# Autodesk Inventor assembly: Ensamblaje Bomba
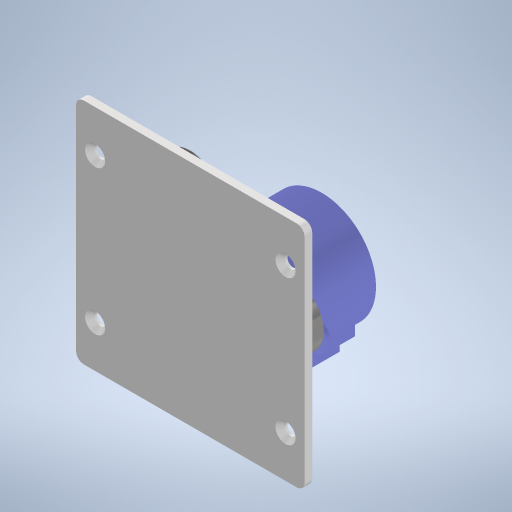
[picture p0: Inventor's stored thumbnail of the model, 512x512]
Saved by Autodesk Inventor 2023 (Build 270158000, 158)
## iProperties
Created: 2023-04-01
Part Number: Ensamblaje Bomba
Document SubType Name: Assembly
Designer: sergi
Author: sergi
## Documents named in this file (7)
- C:\Users\sergi\OneDrive\Escritorio\Objetos 3d\Bomba Persitaltica\Ensamblaje Bomba.iam
- C:\Users\sergi\OneDrive\Escritorio\Objetos 3d\Bomba Persitaltica\Imported Components\stepper_28byj-48\stepper_28byj-48.ipt
- C:\Users\sergi\OneDrive\Escritorio\Objetos 3d\Bomba Persitaltica\Soporte rodamientos.ipt
- C:\Users\sergi\OneDrive\Escritorio\Objetos 3d\Bomba Persitaltica\Rodamiento.ipt
- C:\Users\sergi\OneDrive\Escritorio\Objetos 3d\Bomba Persitaltica\Tapa Soporte rodamientos.ipt
- C:\Users\sergi\OneDrive\Escritorio\Objetos 3d\Bomba Persitaltica\Base.ipt
- C:\Users\sergi\OneDrive\Escritorio\Objetos 3d\Bomba Persitaltica\Tapa.ipt
## Components (8 placed, 6 different names)
1. stepper_28byj-48:1 — Coincidencia:9
2. Soporte rodamientos:1 — Coincidencia:5, Coincidencia:6, Coincidencia:7, Nivelación:1, Nivelación:2, Nivelación:3, Coincidencia:8, Coincidencia:10
3. Rodamiento:1 — Coincidencia:7, Nivelación:1
4. Rodamiento:2 — Coincidencia:5, Nivelación:2
5. Rodamiento:3 — Coincidencia:6, Nivelación:3
6. Tapa Soporte rodamientos:1 — Coincidencia:8
7. Base:1 — Coincidencia:9, Coincidencia:10, Nivelación:4
8. Tapa:1 — Nivelación:4
## Relationships (10: Mate 6, Flush 4)
- Coincidencia:5 [Mate]: Soporte rodamientos:1 ↔ Rodamiento:2
- Coincidencia:6 [Mate]: Soporte rodamientos:1 ↔ Rodamiento:3
- Coincidencia:7 [Mate]: Soporte rodamientos:1 ↔ Rodamiento:1
- Nivelación:1 [Flush]: Soporte rodamientos:1 ↔ Rodamiento:1
- Nivelación:2 [Flush]: Soporte rodamientos:1 ↔ Rodamiento:2
- Nivelación:3 [Flush]: Soporte rodamientos:1 ↔ Rodamiento:3
- Coincidencia:8 [Mate]: Soporte rodamientos:1 ↔ Tapa Soporte rodamientos:1
- Coincidencia:9 [Mate]: stepper_28byj-48:1 ↔ Base:1
- Coincidencia:10 [Mate]: Soporte rodamientos:1 ↔ Base:1
- Nivelación:4 [Flush]: Base:1 ↔ Tapa:1
